# Autodesk Inventor assembly: Assembly1
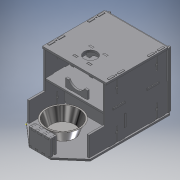
[picture p0: Inventor's stored thumbnail of the model, 180x180]
Saved by Autodesk Inventor 2018 (Build 220112000, 112)
## iProperties
Created: 2018-03-27
Part Number: Assembly1
Document SubType Name: Assembly
Designer: guita
Author: guita
## Documents named in this file (11)
- C:\Users\guita\Documents\ACF\v2.1\Assembly1.iam
- C:\Users\guita\Documents\ACF\v2.1\base.ipt
- C:\Users\guita\Documents\ACF\v2.1\sidewall.ipt
- C:\Users\guita\Documents\ACF\v2.1\bowl-2.ipt
- C:\Users\guita\Documents\ACF\v2.1\front-flat.ipt
- C:\Users\guita\Documents\ACF\v2.1\spacer-1.ipt
- C:\Users\guita\Documents\ACF\v2.1\mid_floor.ipt
- C:\Users\guita\Documents\ACF\v2.1\auger_holder.ipt
- C:\Users\guita\Documents\ACF\v2.1\top.ipt
- C:\Users\guita\Documents\ACF\v2.1\back.ipt
- C:\Users\guita\Documents\ACF\v2.1\lower_front_wall.ipt
## Components (15 placed, 10 different names)
1. base:1 — Mate:1, Mate:2, Mate:3, Mate:4, Mate:5, Mate:6, Mate:7, Mate:8, Mate:9
2. sidewall:1 — Mate:1, Mate:2, Mate:3, Mate:31, Mate:32, Mate:33, Mate:34
3. sidewall:2 — Mate:4, Mate:5, Mate:6, Mate:16, Mate:17, Mate:18, Mate:35, Mate:36, Mate:37, Mate:38, Mate:39, Mate:40
4. bowl-2:1
5. front-flat:1 — Mate:7, Mate:8, Mate:9, Mate:10, Mate:11, Mate:12
6. spacer-1:1 — Mate:10, Mate:11, Mate:12, Mate:13, Mate:14, Mate:15
7. front-flat:2 — Mate:13, Mate:14, Mate:15
8. mid_floor:1 — Mate:16, Mate:17, Mate:18, Mate:19, Mate:20, Mate:21, Mate:22, Mate:23, Mate:24
9. auger_holder:1 — Mate:19, Mate:20, Mate:23
10. auger_holder:2 — Mate:21, Mate:22, Mate:24
11. top:1 — Mate:25, Mate:26, Mate:27, Mate:28, Mate:29, Mate:30, Mate:31, Mate:32, Mate:33
12. auger_holder:3 — Mate:28, Mate:29, Mate:30
13. auger_holder:4 — Mate:25, Mate:26, Mate:27
14. back:1 — Mate:34, Mate:35, Mate:36, Mate:37
15. lower_front_wall:1 — Mate:38, Mate:39, Mate:40
## Relationships (40: Mate 40)
- Mate:1: base:1 ↔ sidewall:1
- Mate:2: base:1 ↔ sidewall:1
- Mate:3: base:1 ↔ sidewall:1
- Mate:4: base:1 ↔ sidewall:2
- Mate:5: base:1 ↔ sidewall:2
- Mate:6: base:1 ↔ sidewall:2
- Mate:7: base:1 ↔ front-flat:1
- Mate:8: base:1 ↔ front-flat:1
- Mate:9: base:1 ↔ front-flat:1
- Mate:10: front-flat:1 ↔ spacer-1:1
- Mate:11: front-flat:1 ↔ spacer-1:1
- Mate:12: front-flat:1 ↔ spacer-1:1
- Mate:13: spacer-1:1 ↔ front-flat:2
- Mate:14: spacer-1:1 ↔ front-flat:2
- Mate:15: spacer-1:1 ↔ front-flat:2
- Mate:16: sidewall:2 ↔ mid_floor:1
- Mate:17: sidewall:2 ↔ mid_floor:1
- Mate:18: sidewall:2 ↔ mid_floor:1
- Mate:19: mid_floor:1 ↔ auger_holder:1
- Mate:20: mid_floor:1 ↔ auger_holder:1
- Mate:21: mid_floor:1 ↔ auger_holder:2
- Mate:22: mid_floor:1 ↔ auger_holder:2
- Mate:23: mid_floor:1 ↔ auger_holder:1
- Mate:24: mid_floor:1 ↔ auger_holder:2
- Mate:25: top:1 ↔ auger_holder:4
- Mate:26: top:1 ↔ auger_holder:4
- Mate:27: top:1 ↔ auger_holder:4
- Mate:28: top:1 ↔ auger_holder:3
- Mate:29: top:1 ↔ auger_holder:3
- Mate:30: top:1 ↔ auger_holder:3
- Mate:31: sidewall:1 ↔ top:1
- Mate:32: sidewall:1 ↔ top:1
- Mate:33: sidewall:1 ↔ top:1
- Mate:34: sidewall:1 ↔ back:1
- Mate:35: sidewall:2 ↔ back:1
- Mate:36: sidewall:2 ↔ back:1
- Mate:37: sidewall:2 ↔ back:1
- Mate:38: sidewall:2 ↔ lower_front_wall:1
- Mate:39: sidewall:2 ↔ lower_front_wall:1
- Mate:40: sidewall:2 ↔ lower_front_wall:1
